# Autodesk Inventor assembly: Quad wring axis
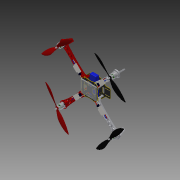
[picture p0: Inventor's stored thumbnail of the model, 180x180]
Saved by Autodesk Inventor 2015 (Build 190159000, 159)
## iProperties
Created: 2015-06-20
Part Number: Quad wring axis
Document SubType Name: Assembly
Designer: Benjamin
Mass: 1060.83 g
Surface Area: 3106.6 cm^2
Volume: 458.713 cm^3
Density: 2.31262 g/cm^3
Author: Benjamin
## Documents named in this file (12)
- C:\Users\Benjamin\Desktop\Kristian\Quad wring axis.iam
- C:\Users\Benjamin\Desktop\Kristian\F450 arm.ipt
- C:\Users\Benjamin\Desktop\Kristian\Imported Components\F450 chasis\F450 chasis.ipt
- C:\Users\Benjamin\Desktop\Kristian\Imported Components\F450 Top Plate\F450 Top Plate.ipt
- C:\Users\Benjamin\Desktop\Kristian\SunnySky X2212_13_980kV.iam
- C:\Users\Benjamin\Desktop\Kristian\Motor\Assemblies\Imported Components\10x4.7-clockwise-propeller\10x4.7-clockwise-propeller.ipt
- C:\Users\Benjamin\Desktop\Kristian\Motor\Assemblies\Imported Components\10x4.7-counterclockwise-propeller\10x4.7-counterclockwise-propeller.ipt
- C:\Users\Benjamin\Desktop\Kristian\Motor\Assemblies\Imported Components\10x4.7-clockwise-propeller\10x4.7-clockwise-propeller_MIR.ipt
- C:\Users\Benjamin\Desktop\Kristian\Motor\Assemblies\Imported Components\10x4.7-counterclockwise-propeller\10x4.7-counterclockwise-propeller_MIR.ipt
- C:\Users\Benjamin\Desktop\Kristian\Motor\Assemblies\Imported Components\Hobby King 20A ESC 3A UBEC\Hobby King 20A ESC 3A UBEC.ipt
- C:\Users\Benjamin\Desktop\Kristian\Flight controller.ipt
- C:\Users\Benjamin\Desktop\Kristian\Batteri.ipt
## Components (20 placed, 11 different names)
1. F450 Top Plate:1 — Mate:1, Mate:2, Mate:3, Flush:5, Mate:18
2. F450 chasis:1 — Mate:4, Flush:4, Mate:5, Mate:20
3. 10x4.7-clockwise-propeller:1 — Mate:11, Mate:12
4. 10x4.7-counterclockwise-propeller:1 — Mate:9, Mate:10
5. 10x4.7-clockwise-propeller_MIR:1 — Mate:13, Mate:14
6. 10x4.7-counterclockwise-propeller_MIR:1 — Mate:15, Mate:16
7. Flight controller:1 — Mate:18, Flush:7, Mate:19
8. Batteri:1 — Mate:20, Flush:8, Flush:9
9. F450 arm:1 — Mate:1, Mate:2, Mate:3, Mate:4
10. F450 arm:2 — Mate:6, Mate:7
11. F450 arm:3
12. F450 arm:4 — Mate:17, Angle:2, Flush:6
13. SunnySky X2212_13_980kV:2 [sub-assembly] — Mate:6, Mate:7, Angle:1, Mate:13, Mate:14
14. SunnySky X2212_13_980kV:3 [sub-assembly] — Mate:9, Mate:11, Mate:12
15. SunnySky X2212_13_980kV:4 [sub-assembly] — Mate:10
16. SunnySky X2212_13_980kV:5 [sub-assembly] — Mate:15, Mate:16
17. Hobby King 20A ESC 3A UBEC:1 — Mate:17, Angle:2, Flush:5, Flush:6
18. Hobby King 20A ESC 3A UBEC:2
19. Hobby King 20A ESC 3A UBEC:3
20. Hobby King 20A ESC 3A UBEC:4
## Component patterns: (4 elements, first: F450 arm:1), (4 elements, first: SunnySky X2212_13_980kV:2), (4 elements, first: Hobby King 20A ESC 3A UBEC:1)
## Relationships (27: Mate 19, Flush 6, Angle 2)
- Mate:1: F450 Top Plate:1 ↔ F450 arm:1
- Mate:2: F450 Top Plate:1 ↔ F450 arm:1
- Mate:3: F450 Top Plate:1 ↔ F450 arm:1
- Mate:4: F450 chasis:1 ↔ F450 arm:1
- Flush:4: F450 chasis:1
- Mate:5: F450 chasis:1
- Mate:6: F450 arm:2 ↔ SunnySky X2212_13_980kV:2
- Mate:7: F450 arm:2 ↔ SunnySky X2212_13_980kV:2
- Angle:1 (-135 deg): SunnySky X2212_13_980kV:2
- Mate:9: 10x4.7-counterclockwise-propeller:1 ↔ SunnySky X2212_13_980kV:3
- Mate:10: 10x4.7-counterclockwise-propeller:1 ↔ SunnySky X2212_13_980kV:4
- Mate:11: 10x4.7-clockwise-propeller:1 ↔ SunnySky X2212_13_980kV:3
- Mate:12: 10x4.7-clockwise-propeller:1 ↔ SunnySky X2212_13_980kV:3
- Mate:13: 10x4.7-clockwise-propeller_MIR:1 ↔ SunnySky X2212_13_980kV:2
- Mate:14: 10x4.7-clockwise-propeller_MIR:1 ↔ SunnySky X2212_13_980kV:2
- Mate:15: 10x4.7-counterclockwise-propeller_MIR:1 ↔ SunnySky X2212_13_980kV:5
- Mate:16: 10x4.7-counterclockwise-propeller_MIR:1 ↔ SunnySky X2212_13_980kV:5
- Mate:17: F450 arm:4 ↔ Hobby King 20A ESC 3A UBEC:1
- Angle:2 (180 deg): F450 arm:4 ↔ Hobby King 20A ESC 3A UBEC:1
- Flush:5 (45 mm): F450 Top Plate:1 ↔ Hobby King 20A ESC 3A UBEC:1
- Flush:6: F450 arm:4 ↔ Hobby King 20A ESC 3A UBEC:1
- Mate:18: F450 Top Plate:1 ↔ Flight controller:1
- Flush:7: Flight controller:1
- Mate:19: Flight controller:1
- Mate:20: F450 chasis:1 ↔ Batteri:1
- Flush:8: Batteri:1
- Flush:9: Batteri:1
